# Autodesk Inventor assembly: reka
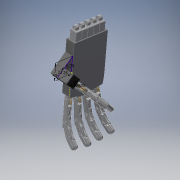
[picture p0: Inventor's stored thumbnail of the model, 180x180]
Saved by Autodesk Inventor 2019 (Build 230136000, 136)
## iProperties
Created: 2019-11-29
Part Number: reka
Material: Ogólny
Document SubType Name: Assembly
Designer: wojta
Author: wojta
## Documents named in this file (9)
- C:\Users\wojta\Desktop\rekav2\reka.iam
- C:\Users\wojta\Desktop\rekav2\dlon\dlon.iam
- C:\Users\wojta\Desktop\rekav2\serwo\Linear actuator v12_MIR_MIR1_MIR.iam
- C:\Users\wojta\Desktop\rekav2\palec\palec.iam
- C:\Users\wojta\Desktop\rekav2\kciuk\kciuk.iam
- C:\Users\wojta\Desktop\rekav2\dlon\prowadzenie.iam
- C:\Users\wojta\Desktop\rekav2\dlon\prowadzenie2.iam
- C:\Users\wojta\Desktop\rekav2\dlon\lozysko.ipt
- C:\Users\wojta\Desktop\rekav2\dlon\nit.ipt
## Components (20 placed, 9 different names)
1. dlon:1 [sub-assembly] — Zestawiający:1, Zestawiający:2, Zestawiający:3, Zestawiający:4, Zestawiający:5, Obrotowe:1, Zestawiający:6, Zestawiający:7, Zestawiający:8, Zestawiający:9, Zestawiający:10, Zestawiający:11, Zestawiający:12, Zestawiający:13, Zestawiający:14, Zestawiający:27, Zestawiający:28, Zestawiający:29, Zestawiający:36, Styczny:1, Styczny:2, Zestawiający:37, Zestawiający:38, Zestawiający:39, Zestawiający:40, Zestawiający:41, Zestawiający:42, Zestawiający:43, Równoległy:9, Równoległy:10, Zestawiający:46, Zestawiający:47
2. Linear actuator v12:1 [sub-assembly] — Zestawiający:23, Równoległy:4, Zestawiający:24, Zestawiający:34, Równoległy:7, Zestawiający:35
3. palec:4 [sub-assembly] — Zestawiający:4, Zestawiający:5, Obrotowe:1
4. palec:3 [sub-assembly] — Zestawiający:3, Zestawiający:6, Zestawiający:9
5. palec:2 [sub-assembly] — Zestawiający:2, Zestawiający:7, Zestawiający:10
6. palec:1 [sub-assembly] — Zestawiający:1, Zestawiający:8, Zestawiający:11
7. kciuk:1 [sub-assembly] — Zestawiający:12, Zestawiający:13, Zestawiający:14
8. Linear actuator v12_MIR_MIR1_MIR:2 [sub-assembly] — Zestawiający:23, Równoległy:4, Zestawiający:24, Zestawiający:27, Zestawiający:28
9. Linear actuator v12_MIR_MIR1_MIR:3 [sub-assembly] — Zestawiający:29, Równoległy:6, Zestawiający:32, Zestawiający:33
10. Linear actuator v12_MIR_MIR1_MIR:4 [sub-assembly] — Zestawiający:30, Zestawiający:31, Równoległy:5, Równoległy:6, Zestawiający:32
11. Linear actuator v12_MIR_MIR1_MIR:5 [sub-assembly] — Zestawiający:30, Zestawiający:31, Równoległy:5, Zestawiający:33, Zestawiający:34, Równoległy:7, Zestawiający:35
12. prowadzenie:1 [sub-assembly] — Zestawiający:36, Styczny:1, Styczny:2, Styczny:3, Styczny:6
13. prowadzenie2:1 [sub-assembly] — Zestawiający:37, Zestawiający:38, Zestawiający:39, Równoległy:8
14. prowadzenie2:2 [sub-assembly] — Zestawiający:40, Zestawiający:41, Równoległy:8, Zestawiający:44
15. prowadzenie2:3 [sub-assembly] — Zestawiający:43, Zestawiający:45, Równoległy:10, Styczny:5
16. prowadzenie2:4 [sub-assembly] — Zestawiający:42, Równoległy:9, Zestawiający:44, Zestawiający:45, Styczny:4
17. lozysko:1 — Zestawiający:46, Styczny:3, Styczny:4, Zestawiający:50, Zestawiający:51
18. lozysko:2 — Zestawiający:47, Styczny:5, Styczny:6, Zestawiający:48, Zestawiający:49
19. nit:1 — Zestawiający:48, Zestawiający:49
20. nit:2 — Zestawiający:50, Zestawiający:51
## Relationships (55: Mate 41, Flush 7, Tangent 6, RevoluteJoint 1)
- Zestawiający:1 [Mate]: dlon:1 ↔ palec:1
- Zestawiający:2 [Mate]: dlon:1 ↔ palec:2
- Zestawiający:3 [Mate]: dlon:1 ↔ palec:3
- Zestawiający:4 [Mate]: dlon:1 ↔ palec:4
- Zestawiający:5 [Mate]: dlon:1 ↔ palec:4
- Obrotowe:1 [RevoluteJoint]: dlon:1 ↔ palec:4
- Zestawiający:6 [Mate]: dlon:1 ↔ palec:3
- Zestawiający:7 [Mate]: dlon:1 ↔ palec:2
- Zestawiający:8 [Mate]: dlon:1 ↔ palec:1
- Zestawiający:9 [Mate]: dlon:1 ↔ palec:3
- Zestawiający:10 [Mate]: dlon:1 ↔ palec:2
- Zestawiający:11 [Mate]: dlon:1 ↔ palec:1
- Zestawiający:12 [Mate]: dlon:1 ↔ kciuk:1
- Zestawiający:13 [Mate]: dlon:1 ↔ kciuk:1
- Zestawiający:14 [Mate]: dlon:1 ↔ kciuk:1
- Zestawiający:23 [Mate]: Linear actuator v12:1 ↔ Linear actuator v12_MIR_MIR1_MIR:2
- Równoległy:4 [Flush]: Linear actuator v12:1 ↔ Linear actuator v12_MIR_MIR1_MIR:2
- Zestawiający:24 [Mate]: Linear actuator v12:1 ↔ Linear actuator v12_MIR_MIR1_MIR:2
- Zestawiający:27 [Mate]: dlon:1 ↔ Linear actuator v12_MIR_MIR1_MIR:2
- Zestawiający:28 [Mate]: dlon:1 ↔ Linear actuator v12_MIR_MIR1_MIR:2
- Zestawiający:29 [Mate]: dlon:1 ↔ Linear actuator v12_MIR_MIR1_MIR:3
- Zestawiający:30 [Mate]: Linear actuator v12_MIR_MIR1_MIR:4 ↔ Linear actuator v12_MIR_MIR1_MIR:5
- Zestawiający:31 [Mate]: Linear actuator v12_MIR_MIR1_MIR:4 ↔ Linear actuator v12_MIR_MIR1_MIR:5
- Równoległy:5 [Flush]: Linear actuator v12_MIR_MIR1_MIR:4 ↔ Linear actuator v12_MIR_MIR1_MIR:5
- Równoległy:6 [Flush]: Linear actuator v12_MIR_MIR1_MIR:3 ↔ Linear actuator v12_MIR_MIR1_MIR:4
- Zestawiający:32 [Mate]: Linear actuator v12_MIR_MIR1_MIR:3 ↔ Linear actuator v12_MIR_MIR1_MIR:4
- Zestawiający:33 [Mate]: Linear actuator v12_MIR_MIR1_MIR:3 ↔ Linear actuator v12_MIR_MIR1_MIR:5
- Zestawiający:34 [Mate]: Linear actuator v12:1 ↔ Linear actuator v12_MIR_MIR1_MIR:5
- Równoległy:7 [Flush]: Linear actuator v12:1 ↔ Linear actuator v12_MIR_MIR1_MIR:5
- Zestawiający:35 [Mate]: Linear actuator v12:1 ↔ Linear actuator v12_MIR_MIR1_MIR:5
- Zestawiający:36 [Mate]: dlon:1 ↔ prowadzenie:1
- Styczny:1 [Tangent]: dlon:1 ↔ prowadzenie:1
- Styczny:2 [Tangent]: dlon:1 ↔ prowadzenie:1
- Zestawiający:37 [Mate] (0.015 mm): dlon:1 ↔ prowadzenie2:1
- Zestawiający:38 [Mate]: dlon:1 ↔ prowadzenie2:1
- Zestawiający:39 [Mate]: dlon:1 ↔ prowadzenie2:1
- Zestawiający:40 [Mate]: dlon:1 ↔ prowadzenie2:2
- Zestawiający:41 [Mate] (2 mm): dlon:1 ↔ prowadzenie2:2
- Równoległy:8 [Flush]: prowadzenie2:1 ↔ prowadzenie2:2
- Zestawiający:42 [Mate]: dlon:1 ↔ prowadzenie2:4
- Zestawiający:43 [Mate]: dlon:1 ↔ prowadzenie2:3
- Równoległy:9 [Flush] (-0.265 mm): dlon:1 ↔ prowadzenie2:4
- Zestawiający:44 [Mate]: prowadzenie2:2 ↔ prowadzenie2:4
- Zestawiający:45 [Mate]: prowadzenie2:3 ↔ prowadzenie2:4
- Równoległy:10 [Flush] (-2.265 mm): dlon:1 ↔ prowadzenie2:3
- Zestawiający:46 [Mate]: dlon:1 ↔ lozysko:1
- Zestawiający:47 [Mate]: dlon:1 ↔ lozysko:2
- Styczny:3 [Tangent]: prowadzenie:1 ↔ lozysko:1
- Styczny:4 [Tangent]: prowadzenie2:4 ↔ lozysko:1
- Styczny:5 [Tangent]: prowadzenie2:3 ↔ lozysko:2
- Styczny:6 [Tangent]: prowadzenie:1 ↔ lozysko:2
- Zestawiający:48 [Mate]: lozysko:2 ↔ nit:1
- Zestawiający:49 [Mate]: lozysko:2 ↔ nit:1
- Zestawiający:50 [Mate]: lozysko:1 ↔ nit:2
- Zestawiający:51 [Mate]: lozysko:1 ↔ nit:2
